# Autodesk Inventor assembly: oczyszczaczPowietrza
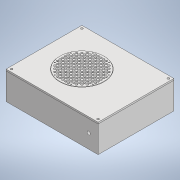
[picture p0: Inventor's stored thumbnail of the model, 180x180]
Saved by Autodesk Inventor 2021 (Build 250183000, 183)
## iProperties
Created: 2021-04-02
Part Number: oczyszczaczPowietrza
Document SubType Name: Assembly
Designer: awitc
Author: awitc
## Documents named in this file (4)
- C:\Users\awitc\Documents\Designed Parts\wentSystem\oczyszczaczPowietrza.iam
- C:\Users\awitc\Documents\Designed Parts\wentSystem\fanCover.ipt
- C:\Users\awitc\Documents\Designed Parts\wentSystem\mainBody.ipt
- C:\Users\awitc\Documents\Designed Parts\wentSystem\back.ipt
## Components (4 placed, 3 different names)
1. fanCover:1 — Insert:4
2. mainBody:1 — Insert:4, Insert:5, Insert:6
3. back:1 — Insert:5, Insert:6, Insert:7
4. fanCover:2 — Insert:7
## Relationships (4: Insert 4)
- Insert:4: fanCover:1 ↔ mainBody:1
- Insert:5: mainBody:1 ↔ back:1
- Insert:6: mainBody:1 ↔ back:1
- Insert:7: back:1 ↔ fanCover:2
